# Autodesk Inventor assembly: neverest 40 + mounts
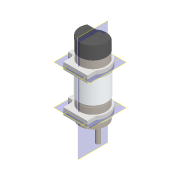
[picture p0: Inventor's stored thumbnail of the model, 180x180]
Saved by Autodesk Inventor 2020 (Build 240168000, 168)
## iProperties
Created: 2020-01-10
Part Number: neverest 40 + mounts
Document SubType Name: Assembly
Designer: ball
Author: ball
## Documents named in this file (3)
- C:\FTC\FTC8863CAD\2019 Robot\Collection\neverest 40 + mounts.iam
- C:\FTC\FTC8863CAD\Actobotics\555 parts\555116 assembly.ipt
- C:\FTC\FTC8863CAD\Andymark\am-2964a Neverest Classic 40.ipt
## Components (3 placed, 2 different names)
1. 555116 assembly:1 — Flush:1, Angle:1
2. 555116 assembly:2 — Mate:2, Mate:3
3. am-2964a Neverest Classic 40:1 — Flush:1, Angle:1, Mate:2, Mate:3
## Relationships (5: Mate 3, Flush 1, Angle 1)
- [Mate]: 555116 assembly:1 ↔ am-2964a Neverest Classic 40:1
- Flush:1 (-8.255 mm): 555116 assembly:1 ↔ am-2964a Neverest Classic 40:1
- Angle:1 (180 deg): 555116 assembly:1 ↔ am-2964a Neverest Classic 40:1
- Mate:2: 555116 assembly:2 ↔ am-2964a Neverest Classic 40:1
- Mate:3: 555116 assembly:2 ↔ am-2964a Neverest Classic 40:1
